# Autodesk Inventor assembly: goniometer_stage
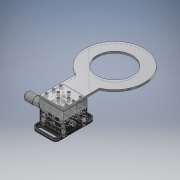
[picture p0: Inventor's stored thumbnail of the model, 180x180]
Saved by Autodesk Inventor 2016 (Build 200138000, 138)
## iProperties
Created: 2017-01-09
Part Number: goniometer_stage
Document SubType Name: Assembly
Designer: stephenholtz
Author: stephenholtz
## Documents named in this file (5)
- \\Mac\AllFiles\Users\stephenholtz\fly-design-files\physiology-stages\goniometer-stage-v01\goniometer_stage.iam
- \\Mac\AllFiles\Users\stephenholtz\fly-design-files\physiology-stages\goniometer-stage-v01\goniometer_stage_standoff_v1.ipt
- \\Mac\AllFiles\Users\stephenholtz\fly-design-files\physiology-stages\goniometer-stage-v01\goniometer_stage_shim_v1.ipt
- \\Mac\AllFiles\Users\stephenholtz\fly-design-files\physiology-stages\goniometer-stage-v01\goniometer_stage_top_v1.ipt
- \\Mac\AllFiles\Users\stephenholtz\fly-design-files\physiology-stages\goniometer-stage-v01\GNL10-Solidworks.ipt
## Components (5 placed, 4 different names)
1. goniometer_stage_standoff_v1:1 — Insert:1, Mate:1, Mate:2, Mate:4, Mate:5
2. goniometer_stage_shim_v1:1 — Insert:1, Insert:2, Mate:2
3. goniometer_stage_shim_v1:2 — Insert:2, Insert:3, Mate:3
4. goniometer_stage_top_v1:1 — Insert:3, Mate:3, Mate:6, Mate:7
5. GNL10-Solidworks:1 — Mate:1, Mate:4, Mate:5
## Relationships (10: Mate 7, Insert 3)
- Insert:1: goniometer_stage_standoff_v1:1 ↔ goniometer_stage_shim_v1:1
- Insert:2: goniometer_stage_shim_v1:1 ↔ goniometer_stage_shim_v1:2
- Insert:3: goniometer_stage_shim_v1:2 ↔ goniometer_stage_top_v1:1
- Mate:1: goniometer_stage_standoff_v1:1 ↔ GNL10-Solidworks:1
- Mate:2: goniometer_stage_standoff_v1:1 ↔ goniometer_stage_shim_v1:1
- Mate:3: goniometer_stage_shim_v1:2 ↔ goniometer_stage_top_v1:1
- Mate:4: goniometer_stage_standoff_v1:1 ↔ GNL10-Solidworks:1
- Mate:5: goniometer_stage_standoff_v1:1 ↔ GNL10-Solidworks:1
- Mate:6: goniometer_stage_top_v1:1
- Mate:7: goniometer_stage_top_v1:1
